# Autodesk Inventor assembly: Beginning_assembly
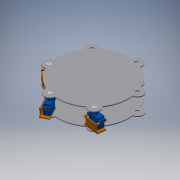
[picture p0: Inventor's stored thumbnail of the model, 180x180]
Saved by Autodesk Inventor 2016 (Build 200138000, 138)
## iProperties
Created: 2015-10-08
Part Number: Beginning_assembly
Document SubType Name: Assembly
Designer: powasar16
Author: powasar16
## Documents named in this file (6)
- C:\Users\powasar16\Documents\GitHub\SpyderRobot\Inventor\Created Parts\Beginning_assembly.iam
- C:\Users\powasar16\Documents\GitHub\SpyderRobot\Inventor\Created Parts\Arduino.ipt
- C:\Users\powasar16\Documents\GitHub\SpyderRobot\Inventor\Created Parts\Base_bottom.ipt
- C:\Users\powasar16\Documents\GitHub\SpyderRobot\Inventor\Imported Parts\Motherboard Standoff 12mm M3x0.5.ipt
- C:\Users\powasar16\Documents\GitHub\SpyderRobot\Inventor\Created Parts\Servo_vice.ipt
- C:\Users\powasar16\Documents\GitHub\SpyderRobot\Inventor\Created Parts\Servo.iam
## Components (17 placed, 5 different names)
1. Arduino:1 — Mate:2, Mate:3, Mate:4, Mate:5, Mate:14, Mate:15, Mate:16, Mate:17, Mate:18, Mate:19, Mate:20, Mate:21, Mate:22
2. Base_bottom:1 — Mate:2, Mate:3, Mate:4, Mate:5, Mate:6, Mate:7, Mate:8, Mate:9, Mate:10, Mate:11, Mate:12, Mate:13, Mate:23, Mate:24, Mate:28, Mate:29
3. Motherboard Standoff 12mm M3x0.5:1 — Mate:7, Mate:12
4. Motherboard Standoff 12mm M3x0.5:2 — Mate:6, Mate:11, Mate:14
5. Motherboard Standoff 12mm M3x0.5:3 — Mate:9, Mate:13
6. Motherboard Standoff 12mm M3x0.5:4 — Mate:8, Mate:10
7. Motherboard Standoff 12mm M3x0.5:5 — Mate:15, Mate:16
8. Motherboard Standoff 12mm M3x0.5:6 — Mate:21, Mate:22
9. Motherboard Standoff 12mm M3x0.5:7 — Mate:19, Mate:20
10. Motherboard Standoff 12mm M3x0.5:8 — Mate:17, Mate:18
11. Base_bottom:2 — Mate:23, Mate:24, Flush:1, Mate:36, Flush:2, Flush:3, Mate:37
12. Servo_vice:1 — Mate:25, Mate:26, Mate:27, Mate:29
13. Servo:1 [sub-assembly] — Mate:25, Mate:26, Mate:27, Mate:28, Flush:1
14. Servo_vice:2
15. Servo:2 [sub-assembly] — Mate:36, Flush:2
16. Servo_vice:3
17. Servo:3 [sub-assembly] — Flush:3, Mate:37
## Relationships (39: Mate 36, Flush 3)
- Mate:2: Arduino:1 ↔ Base_bottom:1
- Mate:3: Arduino:1 ↔ Base_bottom:1
- Mate:4: Arduino:1 ↔ Base_bottom:1
- Mate:5: Arduino:1 ↔ Base_bottom:1
- Mate:6: Base_bottom:1 ↔ Motherboard Standoff 12mm M3x0.5:2
- Mate:7: Base_bottom:1 ↔ Motherboard Standoff 12mm M3x0.5:1
- Mate:8: Base_bottom:1 ↔ Motherboard Standoff 12mm M3x0.5:4
- Mate:9: Base_bottom:1 ↔ Motherboard Standoff 12mm M3x0.5:3
- Mate:10: Base_bottom:1 ↔ Motherboard Standoff 12mm M3x0.5:4
- Mate:11: Base_bottom:1 ↔ Motherboard Standoff 12mm M3x0.5:2
- Mate:12: Base_bottom:1 ↔ Motherboard Standoff 12mm M3x0.5:1
- Mate:13: Base_bottom:1 ↔ Motherboard Standoff 12mm M3x0.5:3
- Mate:14: Arduino:1 ↔ Motherboard Standoff 12mm M3x0.5:2
- Mate:15: Arduino:1 ↔ Motherboard Standoff 12mm M3x0.5:5
- Mate:16: Arduino:1 ↔ Motherboard Standoff 12mm M3x0.5:5
- Mate:17: Arduino:1 ↔ Motherboard Standoff 12mm M3x0.5:8
- Mate:18: Arduino:1 ↔ Motherboard Standoff 12mm M3x0.5:8
- Mate:19: Arduino:1 ↔ Motherboard Standoff 12mm M3x0.5:7
- Mate:20: Arduino:1 ↔ Motherboard Standoff 12mm M3x0.5:7
- Mate:21: Arduino:1 ↔ Motherboard Standoff 12mm M3x0.5:6
- Mate:22: Arduino:1 ↔ Motherboard Standoff 12mm M3x0.5:6
- Mate:23: Base_bottom:1 ↔ Base_bottom:2
- Mate:24: Base_bottom:1 ↔ Base_bottom:2
- Mate:25: Servo_vice:1 ↔ Servo:1
- Mate:26: Servo_vice:1 ↔ Servo:1
- Mate:27: Servo_vice:1 ↔ Servo:1
- Mate:28: Base_bottom:1 ↔ Servo:1
- Mate:29 (1.905 mm): Base_bottom:1 ↔ Servo_vice:1
- Flush:1: Base_bottom:2 ↔ Servo:1
- [Mate]: Servo_vice:2 ↔ Servo:2
- [Mate]: Servo_vice:2 ↔ Servo:2
- [Mate]: Servo_vice:2 ↔ Servo:2
- [Mate]: Servo_vice:3 ↔ Servo:3
- [Mate]: Servo_vice:3 ↔ Servo:3
- [Mate]: Servo_vice:3 ↔ Servo:3
- Mate:36: Base_bottom:2 ↔ Servo:2
- Flush:2: Base_bottom:2 ↔ Servo:2
- Flush:3: Base_bottom:2 ↔ Servo:3
- Mate:37: Base_bottom:2 ↔ Servo:3
## Named parameters: d32_d26 = 0 mm, d33_d27 = 0 mm, d34_d28 = 0 mm, d35_d26 = 0 mm, d36_d27 = 0 mm, d37_d28 = 0 mm
